# Autodesk Inventor assembly: kbd
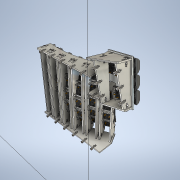
[picture p0: Inventor's stored thumbnail of the model, 180x180]
Saved by Autodesk Inventor 2020.1 (Build 241239000, 239)
## iProperties
Created: 2019-07-12
Part Number: kbd
Document SubType Name: Assembly
Designer: Thibault
Author: Thibault
## Documents named in this file (6)
- C:\Users\Thibault Polge\Documents\Habilis\mech\kbd.iam
- C:\Users\Thibault Polge\Documents\Habilis\mech\keywell.iam
- C:\Users\Thibault Polge\Documents\Habilis\mech\tc_switchplate.iam
- C:\Users\Thibault Polge\Documents\Habilis\mech\base_plate.ipt
- C:\Users\Thibault Polge\Documents\Habilis\mech\shared_parameters.ipt
- C:\Users\Thibault Polge\Documents\Inventor\Content Center Files\R2020\fr-FR\BS 4168(1)\BS 4168 - M2 x 8(1).ipt
## Components (21 placed, 4 different names)
1. base_plate:1 — Affleurement:5, Placage:1, Placage:2, Placage:3, Placage:4, Logement:1, Logement:2, Logement:3, Logement:4, Logement:5, Logement:6, Logement:7, Logement:8, Logement:9, Logement:10, Logement:11, Logement:12, Logement:13, Logement:14, Logement:15, Logement:16, Logement:17, Logement:18, Affleurement:6, Affleurement:7, Affleurement:8
2. keywell:1 [sub-assembly] — Affleurement:4, Affleurement:5, Placage:1, Placage:2
3. tc_switchplate:1 [sub-assembly] — Affleurement:4, Placage:3, Placage:4
4. BS 4168 : Pièce 1 Vis cylindrique à six pans creux - Métrique M2 x 8:1 — Logement:1
5. BS 4168 : Pièce 1 Vis cylindrique à six pans creux - Métrique M2 x 8:2 — Logement:2
6. BS 4168 : Pièce 1 Vis cylindrique à six pans creux - Métrique M2 x 8:3 — Logement:3
7. BS 4168 : Pièce 1 Vis cylindrique à six pans creux - Métrique M2 x 8:4 — Logement:4
8. BS 4168 : Pièce 1 Vis cylindrique à six pans creux - Métrique M2 x 8:5 — Logement:5
9. BS 4168 : Pièce 1 Vis cylindrique à six pans creux - Métrique M2 x 8:6 — Logement:6
10. BS 4168 : Pièce 1 Vis cylindrique à six pans creux - Métrique M2 x 8:7 — Logement:7
11. BS 4168 : Pièce 1 Vis cylindrique à six pans creux - Métrique M2 x 8:8 — Logement:8
12. BS 4168 : Pièce 1 Vis cylindrique à six pans creux - Métrique M2 x 8:9 — Logement:9
13. BS 4168 : Pièce 1 Vis cylindrique à six pans creux - Métrique M2 x 8:10 — Logement:10
14. BS 4168 : Pièce 1 Vis cylindrique à six pans creux - Métrique M2 x 8:11 — Logement:11
15. BS 4168 : Pièce 1 Vis cylindrique à six pans creux - Métrique M2 x 8:12 — Logement:12
16. BS 4168 : Pièce 1 Vis cylindrique à six pans creux - Métrique M2 x 8:13 — Logement:13
17. BS 4168 : Pièce 1 Vis cylindrique à six pans creux - Métrique M2 x 8:14 — Logement:14
18. BS 4168 : Pièce 1 Vis cylindrique à six pans creux - Métrique M2 x 8:15 — Logement:15
19. BS 4168 : Pièce 1 Vis cylindrique à six pans creux - Métrique M2 x 8:16 — Logement:16
20. BS 4168 : Pièce 1 Vis cylindrique à six pans creux - Métrique M2 x 8:17 — Logement:17
21. BS 4168 : Pièce 1 Vis cylindrique à six pans creux - Métrique M2 x 8:18 — Logement:18
## Relationships (27: Insert 18, Flush 5, Mate 4)
- Affleurement:4 [Flush]: keywell:1 ↔ tc_switchplate:1
- Affleurement:5 [Flush]: base_plate:1 ↔ keywell:1
- Placage:1 [Mate] (0.05 mm): base_plate:1 ↔ keywell:1
- Placage:2 [Mate] (0.05 mm): base_plate:1 ↔ keywell:1
- Placage:3 [Mate] (0.05 mm): base_plate:1 ↔ tc_switchplate:1
- Placage:4 [Mate] (0.05 mm): base_plate:1 ↔ tc_switchplate:1
- Logement:1 [Insert]: base_plate:1 ↔ BS 4168 : Pièce 1 Vis cylindrique à six pans creux - Métrique M2 x 8:1
- Logement:2 [Insert]: base_plate:1 ↔ BS 4168 : Pièce 1 Vis cylindrique à six pans creux - Métrique M2 x 8:2
- Logement:3 [Insert]: base_plate:1 ↔ BS 4168 : Pièce 1 Vis cylindrique à six pans creux - Métrique M2 x 8:3
- Logement:4 [Insert]: base_plate:1 ↔ BS 4168 : Pièce 1 Vis cylindrique à six pans creux - Métrique M2 x 8:4
- Logement:5 [Insert]: base_plate:1 ↔ BS 4168 : Pièce 1 Vis cylindrique à six pans creux - Métrique M2 x 8:5
- Logement:6 [Insert]: base_plate:1 ↔ BS 4168 : Pièce 1 Vis cylindrique à six pans creux - Métrique M2 x 8:6
- Logement:7 [Insert]: base_plate:1 ↔ BS 4168 : Pièce 1 Vis cylindrique à six pans creux - Métrique M2 x 8:7
- Logement:8 [Insert]: base_plate:1 ↔ BS 4168 : Pièce 1 Vis cylindrique à six pans creux - Métrique M2 x 8:8
- Logement:9 [Insert]: base_plate:1 ↔ BS 4168 : Pièce 1 Vis cylindrique à six pans creux - Métrique M2 x 8:9
- Logement:10 [Insert]: base_plate:1 ↔ BS 4168 : Pièce 1 Vis cylindrique à six pans creux - Métrique M2 x 8:10
- Logement:11 [Insert]: base_plate:1 ↔ BS 4168 : Pièce 1 Vis cylindrique à six pans creux - Métrique M2 x 8:11
- Logement:12 [Insert]: base_plate:1 ↔ BS 4168 : Pièce 1 Vis cylindrique à six pans creux - Métrique M2 x 8:12
- Logement:13 [Insert]: base_plate:1 ↔ BS 4168 : Pièce 1 Vis cylindrique à six pans creux - Métrique M2 x 8:13
- Logement:14 [Insert]: base_plate:1 ↔ BS 4168 : Pièce 1 Vis cylindrique à six pans creux - Métrique M2 x 8:14
- Logement:15 [Insert]: base_plate:1 ↔ BS 4168 : Pièce 1 Vis cylindrique à six pans creux - Métrique M2 x 8:15
- Logement:16 [Insert]: base_plate:1 ↔ BS 4168 : Pièce 1 Vis cylindrique à six pans creux - Métrique M2 x 8:16
- Logement:17 [Insert]: base_plate:1 ↔ BS 4168 : Pièce 1 Vis cylindrique à six pans creux - Métrique M2 x 8:17
- Logement:18 [Insert]: base_plate:1 ↔ BS 4168 : Pièce 1 Vis cylindrique à six pans creux - Métrique M2 x 8:18
- Affleurement:6 [Flush]: base_plate:1
- Affleurement:7 [Flush]: base_plate:1
- Affleurement:8 [Flush]: base_plate:1
## Named parameters: extra_slot_dim = 0.1 mm
